# Autodesk Inventor assembly: Enclosure Assembly
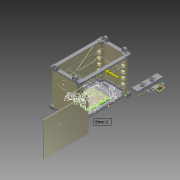
[picture p0: Inventor's stored thumbnail of the model, 180x180]
Saved by Autodesk Inventor 2015 (Build 190159000, 159)
## iProperties
Created: 2015-04-17
Part Number: Enclosure Assembly
Document SubType Name: Assembly
Designer: Akovo_000
Material: NylonD2W
Mass: 325.705 g
Surface Area: 4296.01 cm^2
Volume: 317.981 cm^3
Density: 1.02429 g/cm^3
Author: Akovo_000
## Documents named in this file (18)
- C:\Users\Akovo_000\SkyDrive\3D printing\Enclosure Half-Open\Enclosure Assembly.iam
- C:\Users\Akovo_000\SkyDrive\3D printing\Enclosure Half-Open\NUCholder.ipt
- C:\Users\Akovo_000\SkyDrive\3D printing\Enclosure Half-Open\SidePanelNarrow.ipt
- C:\Users\Akovo_000\SkyDrive\3D printing\Enclosure Half-Open\SidePanelwide.ipt
- C:\Users\Akovo_000\SkyDrive\3D printing\Enclosure Half-Open\SidePanelNarrowWithPowerButton.ipt
- C:\Users\Akovo_000\SkyDrive\3D printing\Enclosure Half-Open\Pillar2.ipt
- C:\Users\Akovo_000\SkyDrive\3D printing\Enclosure Half-Open\GenericPanel.ipt
- C:\Users\Akovo_000\SkyDrive\3D printing\Enclosure Half-Open\CameraCover.ipt
- C:\Users\Akovo_000\SkyDrive\3D printing\Enclosure Half-Open\LensPlane.ipt
- C:\Users\Akovo_000\SkyDrive\3D printing\Enclosure Half-Open\Lid2.ipt
- C:\Users\Akovo_000\SkyDrive\3D printing\Enclosure Half-Open\FilterHolder.ipt
- C:\Users\Akovo_000\SkyDrive\3D printing\Enclosure Half-Open\NutInserperFilling.ipt
- C:\Users\Akovo_000\SkyDrive\3D printing\Enclosure Half-Open\Enclosure Assembly\AIP\FEA\be8m3005c.fins
- C:\Users\Akovo_000\SkyDrive\3D printing\Enclosure Half-Open\Enclosure Assembly\AIP\FEA\be8m30068.fsat
- C:\Users\Akovo_000\SkyDrive\3D printing\Enclosure Half-Open\Enclosure Assembly\AIP\FEA\be8m30074.ftes
- C:\Users\Akovo_000\SkyDrive\3D printing\Enclosure Half-Open\Enclosure Assembly\AIP\FEA\be8m30074.fwiz
- C:\Users\Akovo_000\SkyDrive\3D printing\Enclosure Half-Open\Enclosure Assembly\AIP\FEA\be8m301cw.fmsh
- C:\Users\Akovo_000\SkyDrive\3D printing\Enclosure Half-Open\Enclosure Assembly\AIP\FEA\be8m301ds.fres
## Components (22 placed, 11 different names)
1. Pillar2:1 — Rigid:2, Rigid:6
2. Pillar2:2 — Rigid:4
3. Pillar2:3 — Rigid:5, Slider:1
4. Pillar2:4 — Rigid:3, Slider:2, Slider:3
5. SidePanelNarrowWithPowerButton:1 — Slider:3
6. SidePanelNarrow:1 — Rigid:7
7. SidePanelwide:1
8. SidePanelwide:2 — Slider:1
9. NUCholder:1 — Slider:2
10. GenericPanel:1
11. CameraCover:1 — Rigid:1
12. LensPlane:1 — Rigid:1, Rigid:2, Rigid:3, Rigid:4, Rigid:5
13. Lid2:1 — Rigid:6, Rigid:7
14. FilterHolder:1
15. NutInserperFilling:1
16. NutInserperFilling:2
17. NutInserperFilling:3
18. NutInserperFilling:4
19. NutInserperFilling:5
20. NutInserperFilling:6
21. NutInserperFilling:7
22. NutInserperFilling:8
## Relationships (10: WeldJoint 7, TranslationJoint 3)
- Rigid:1 [WeldJoint]: CameraCover:1 ↔ LensPlane:1
- Rigid:2 [WeldJoint]: Pillar2:1 ↔ LensPlane:1
- Rigid:3 [WeldJoint]: Pillar2:4 ↔ LensPlane:1
- Rigid:4 [WeldJoint]: Pillar2:2 ↔ LensPlane:1
- Rigid:5 [WeldJoint]: Pillar2:3 ↔ LensPlane:1
- Rigid:6 [WeldJoint]: Pillar2:1 ↔ Lid2:1
- Slider:1 [TranslationJoint]: Pillar2:3 ↔ SidePanelwide:2
- Slider:2 [TranslationJoint]: Pillar2:4 ↔ NUCholder:1
- Slider:3 [TranslationJoint]: Pillar2:4 ↔ SidePanelNarrowWithPowerButton:1
- Rigid:7 [WeldJoint]: SidePanelNarrow:1 ↔ Lid2:1
## Named parameters: sa_3 = -5000, sa_4 = -7e-13, sa_5 = 1e-13
note: some values were not read from the file. Shown as the stored number, unit unknown: "sa_3", "sa_4", "sa_5".
